# Autodesk Inventor assembly: full deadbolt controller enclosure assembly
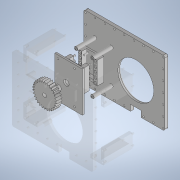
[picture p0: Inventor's stored thumbnail of the model, 180x180]
Saved by Autodesk Inventor 2022 (Build 260153000, 153)
## iProperties
Created: 2022-01-25
Part Number: full deadbolt controller enclosure assembly
Document SubType Name: Assembly
Designer: alecw
Author: alecw
## Documents named in this file (7)
- W:\My Drive\Coding and Projects\smart home\smart-deadbolt\3D Modelling\full deadbolt controller enclosure assembly.iam
- W:\My Drive\Coding and Projects\smart home\smart-deadbolt\3D Modelling\door backplate.ipt
- W:\My Drive\Coding and Projects\smart home\smart-deadbolt\3D Modelling\motor mount plate.iam
- W:\My Drive\Coding and Projects\smart home\smart-deadbolt\3D Modelling\door top plate with window.ipt
- W:\My Drive\Coding and Projects\smart home\smart-deadbolt\3D Modelling\enclosure corner standoffs.ipt
- W:\My Drive\Coding and Projects\smart home\smart-deadbolt\3D Modelling\motor gear.ipt
- W:\My Drive\Coding and Projects\smart home\smart-deadbolt\3D Modelling\motor holder top.ipt
## Components (6 placed, 6 different names)
1. door backplate:1 — Flush:3, Flush:4, Mate:8
2. motor mount plate:1 [sub-assembly] — Mate:1, Mate:2, Mate:3, Mate:4, Mate:5, Mate:6, Mate:9, Mate:10
3. door top plate with window:1 — Mate:1, Mate:2, Mate:3, Mate:7, Flush:1, Flush:2, Flush:3, Flush:4
4. enclosure corner standoffs:1 — Mate:7, Flush:1, Flush:2, Mate:8
5. motor gear:1 — Mate:9, Mate:10
6. motor holder top:1 — Mate:4, Mate:5, Mate:6
## Relationships (14: Mate 10, Flush 4)
- Mate:1 (30 mm): motor mount plate:1 ↔ door top plate with window:1
- Mate:2: motor mount plate:1 ↔ door top plate with window:1
- Mate:3: motor mount plate:1 ↔ door top plate with window:1
- Mate:4: motor mount plate:1 ↔ motor holder top:1
- Mate:5 (15 mm): motor mount plate:1 ↔ motor holder top:1
- Mate:6: motor mount plate:1 ↔ motor holder top:1
- Mate:7 (60 mm): door top plate with window:1 ↔ enclosure corner standoffs:1
- Flush:1: door top plate with window:1 ↔ enclosure corner standoffs:1
- Flush:2: door top plate with window:1 ↔ enclosure corner standoffs:1
- Flush:3: door backplate:1 ↔ door top plate with window:1
- Flush:4: door backplate:1 ↔ door top plate with window:1
- Mate:8 (15 mm): door backplate:1 ↔ enclosure corner standoffs:1
- Mate:9 (30.5 mm): motor mount plate:1 ↔ motor gear:1
- Mate:10: motor mount plate:1 ↔ motor gear:1
